# Autodesk Inventor assembly: electronics_box
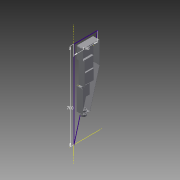
[picture p0: Inventor's stored thumbnail of the model, 180x180]
Saved by Autodesk Inventor 2015 (Build 190159000, 159)
## iProperties
Created: 2015-10-09
Part Number: electronics_box
Description: insert description/title
Document SubType Name: Assembly
Designer: c3132704
Part Category: insert part category and press enter to fill value
Author: c3132704
## Documents named in this file (7)
- C:\Users\c3132704\Documents\GitHub\CAD\electronics_box.iam
- C:\Users\c3132704\Documents\GitHub\CAD\outline.ipt
- C:\Users\c3132704\Documents\GitHub\CAD\stig.ipt
- C:\Users\c3132704\Documents\GitHub\CAD\fart.ipt
- C:\Users\c3132704\Documents\GitHub\CAD\solenoid_dvr.ipt
- C:\Users\c3132704\Documents\GitHub\CAD\BOX.ipt
- C:\Users\c3132704\Documents\GitHub\CAD\Imported Components\c-hd34-24-47pe-a-3d\c-hd34-24-47pe-a-3d.ipt
## Components (7 placed, 6 different names)
1. outline:1
2. stig:1 — Mate:3, Angle:2
3. fart:1 — Mate:4, Angle:1
4. solenoid_dvr:1 — Mate:2
5. solenoid_dvr:2 — Mate:1
6. BOX:1 — Mate:5, Flush:1, Mate:4, Mate:3, Mate:2, Mate:1
7. c-hd34-24-47pe-a-3d:1 — Mate:5, Flush:1
## Relationships (8: Mate 5, Angle 2, Flush 1)
- Mate:1: solenoid_dvr:2 ↔ BOX:1
- Mate:2: solenoid_dvr:1 ↔ BOX:1
- Mate:3: stig:1 ↔ BOX:1
- Mate:4: fart:1 ↔ BOX:1
- Angle:1 (90 deg): fart:1
- Angle:2 (0 deg): stig:1
- Mate:5: BOX:1 ↔ c-hd34-24-47pe-a-3d:1
- Flush:1: BOX:1 ↔ c-hd34-24-47pe-a-3d:1
